# Autodesk Inventor assembly: مهمه 2
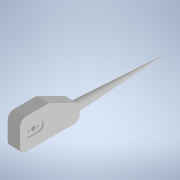
[picture p0: Inventor's stored thumbnail of the model, 180x180]
Saved by Autodesk Inventor 2022 (Build 260153000, 153)
## iProperties
Created: 2021-07-07
Part Number: مهمه 2
Document SubType Name: Assembly
Designer: Nay
Author: Nay
## Documents named in this file (3)
- C:\Users\Nay\OneDrive\المستندات\مهمه 2.iam
- C:\Users\Nay\Downloads\Part1.ipt
- C:\Users\Nay\Downloads\Part2.ipt
## Components (2 placed, 2 different names)
1. Part1:1 — Rigid:1
2. Part2:1 — Rigid:1
## Relationships (1: WeldJoint 1)
- Rigid:1 [WeldJoint]: Part1:1 ↔ Part2:1
